# Autodesk Inventor assembly: ShooterAssemblyV04
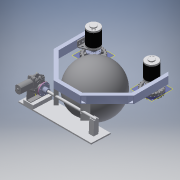
[picture p0: Inventor's stored thumbnail of the model, 180x180]
Saved by Autodesk Inventor 2016 SP1 (Build 200210100, 210)
## iProperties
Created: 2016-02-07
Part Number: ShooterAssemblyV04
Document SubType Name: Assembly
Designer: steele
Author: steele
## Documents named in this file (11)
- C:\snobotics\CAD-Development\robSteele\SnoBotics2016\2016-05-05-ShooterPrototype\ShooterAssemblyV04.iam
- C:\snobotics\CAD-Development\robSteele\SnoBotics2016\2016-05-05-ShooterPrototype\ShooterFrameV02.ipt
- C:\snobotics\CAD-Development\robSteele\SnoBotics2016\DraftOfBoulder.ipt
- C:\snobotics\CAD-Development\robSteele\SnoBotics2016\2016-05-05-ShooterPrototype\Mini_CIM_MotorHub_4_inch_wheel.iam
- C:\snobotics\CAD-Development\robSteele\SnoBotics2016\2016-05-05-ShooterPrototype\postForAxel.ipt
- C:\snobotics\CAD-Development\robSteele\SnoBotics2016\2016-05-05-ShooterPrototype\AluminumRodForShooter.ipt
- C:\snobotics\CAD-Development\robSteele\SnoBotics2016\AM Parts\am-0077a-500 Key Hub r2.ipt
- C:\snobotics\CAD-Development\robSteele\SnoBotics2016\AM Parts\SnowBlowerMotorAndHub.iam
- C:\snobotics\CAD-Development\robSteele\SnoBotics2016\AM Parts\rsSnowBlowerMount.ipt
- C:\snobotics\CAD-Development\robSteele\SnoBotics2016\2016-05-05-ShooterPrototype\SupportPlateToAttachToRobotBase.ipt
- C:\snobotics\CAD-Development\robSteele\SnoBotics2016\2016-05-05-ShooterPrototype\CIM_MotorHub_4_inch_wheel.iam
## Components (11 placed, 10 different names)
1. ShooterFrameV02:1 — Mate:1, Flush:1, Flush:2, Mate:2, Mate:4, Flush:3, Mate:5, Mate:6, Mate:7, Mate:11, Flush:4, Mate:12, Mate:14, Mate:15
2. Mini_CIM_MotorHub_4_inch_wheel:1 [sub-assembly] — Mate:1, Flush:1, Flush:2, Mate:3, Mate:9, Flush:5
3. DraftOfBoulder:1 — Mate:2, Mate:3, Mate:4
4. postForAxel:1 — Flush:3, Mate:5, Mate:6
5. postForAxel:2 — Mate:7, Flush:4, Mate:12
6. AluminumRodForShooter:1 — Mate:9, Mate:10, Mate:11, Insert:1, Insert:4
7. am-0077a-500 Key Hub r2:1 — Insert:1, Insert:2
8. SnowBlowerMotorAndHub:1 [sub-assembly] — Insert:2, Insert:3
9. CIM_MotorHub_4_inch_wheel:1 [sub-assembly] — Mate:14, Mate:15, Flush:5
10. rsSnowBlowerMount:1 — Insert:3, Mate:13
11. SupportPlateToAttachToRobotBase:1 — Insert:4, Mate:13
## Relationships (23: Mate 14, Flush 5, Insert 4)
- Mate:1: ShooterFrameV02:1 ↔ Mini_CIM_MotorHub_4_inch_wheel:1
- Flush:1: ShooterFrameV02:1 ↔ Mini_CIM_MotorHub_4_inch_wheel:1
- Flush:2 (-4.7625 mm): ShooterFrameV02:1 ↔ Mini_CIM_MotorHub_4_inch_wheel:1
- Mate:2: ShooterFrameV02:1 ↔ DraftOfBoulder:1
- Mate:3: Mini_CIM_MotorHub_4_inch_wheel:1 ↔ DraftOfBoulder:1
- Mate:4: ShooterFrameV02:1 ↔ DraftOfBoulder:1
- Flush:3: ShooterFrameV02:1 ↔ postForAxel:1
- Mate:5: ShooterFrameV02:1 ↔ postForAxel:1
- Mate:6: ShooterFrameV02:1 ↔ postForAxel:1
- Mate:7: ShooterFrameV02:1 ↔ postForAxel:2
- Mate:9: Mini_CIM_MotorHub_4_inch_wheel:1 ↔ AluminumRodForShooter:1
- Mate:10: AluminumRodForShooter:1
- Mate:11: ShooterFrameV02:1 ↔ AluminumRodForShooter:1
- Flush:4: ShooterFrameV02:1 ↔ postForAxel:2
- Mate:12: ShooterFrameV02:1 ↔ postForAxel:2
- Insert:1: AluminumRodForShooter:1 ↔ am-0077a-500 Key Hub r2:1
- Insert:2: am-0077a-500 Key Hub r2:1 ↔ SnowBlowerMotorAndHub:1
- Insert:3: SnowBlowerMotorAndHub:1 ↔ rsSnowBlowerMount:1
- Insert:4: AluminumRodForShooter:1 ↔ SupportPlateToAttachToRobotBase:1
- Mate:13: rsSnowBlowerMount:1 ↔ SupportPlateToAttachToRobotBase:1
- Mate:14: ShooterFrameV02:1 ↔ CIM_MotorHub_4_inch_wheel:1
- Mate:15: ShooterFrameV02:1 ↔ CIM_MotorHub_4_inch_wheel:1
- Flush:5: Mini_CIM_MotorHub_4_inch_wheel:1 ↔ CIM_MotorHub_4_inch_wheel:1
